# Autodesk Inventor assembly: Box
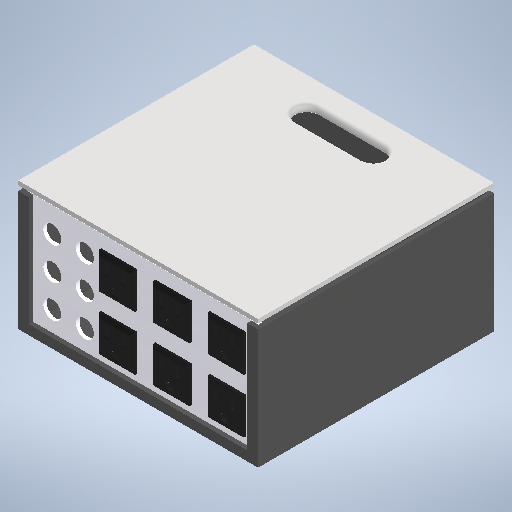
[picture p0: Inventor's stored thumbnail of the model, 512x512]
Saved by Autodesk Inventor 2025 (Build 290162000, 162)
## iProperties
Created: 2024-08-10
Part Number: Box
Document SubType Name: Assembly
Designer: ethan
Author: ethan
## Documents named in this file (5)
- C:\Users\ethan\Documents\GitHub\3D-Pants\AutoFrog\Box.iam
- C:\Users\ethan\Documents\GitHub\3D-Pants\AutoFrog\Box.ipt
- C:\Users\ethan\Documents\GitHub\3D-Pants\AutoFrog\faceplate.ipt
- C:\Users\ethan\Documents\GitHub\3D-Pants\AutoFrog\Plug.ipt
- C:\Users\ethan\Documents\GitHub\3D-Pants\AutoFrog\Lid.ipt
## Components (9 placed, 4 different names)
1. Box:1 — Mate:1, Mate:2, Flush:1, Flush:2
2. faceplate:1 — Mate:1, Mate:2, Mate:3, Mate:5, Mate:6, Mate:7, Mate:8, Mate:9, Mate:10, Mate:11, Mate:12, Mate:13, Mate:14, Mate:15, Mate:16, Mate:17, Mate:18, Mate:19, Mate:20, Mate:21, Mate:22
3. Plug:1 — Mate:8, Mate:9, Mate:10
4. Plug:2 — Mate:5, Mate:11, Mate:19
5. Plug:3 — Mate:7, Mate:13, Mate:18
6. Plug:4 — Mate:14, Mate:17, Mate:21
7. Plug:5 — Mate:6, Mate:15, Mate:16, Mate:22
8. Plug:6 — Mate:3, Mate:12, Mate:20
9. Lid:1 — Flush:1, Flush:2
## Relationships (23: Mate 21, Flush 2)
- Mate:1: Box:1 ↔ faceplate:1
- Mate:2: Box:1 ↔ faceplate:1
- Mate:3: faceplate:1 ↔ Plug:6
- Mate:5: faceplate:1 ↔ Plug:2
- Mate:6: faceplate:1 ↔ Plug:5
- Mate:7: faceplate:1 ↔ Plug:3
- Mate:8: faceplate:1 ↔ Plug:1
- Mate:9: faceplate:1 ↔ Plug:1
- Mate:10: faceplate:1 ↔ Plug:1
- Mate:11: faceplate:1 ↔ Plug:2
- Mate:12: faceplate:1 ↔ Plug:6
- Mate:13: faceplate:1 ↔ Plug:3
- Mate:14: faceplate:1 ↔ Plug:4
- Mate:15: faceplate:1 ↔ Plug:5
- Mate:16: faceplate:1 ↔ Plug:5
- Mate:17: faceplate:1 ↔ Plug:4
- Mate:18: faceplate:1 ↔ Plug:3
- Mate:19: faceplate:1 ↔ Plug:2
- Mate:20: faceplate:1 ↔ Plug:6
- Mate:21: faceplate:1 ↔ Plug:4
- Mate:22: faceplate:1 ↔ Plug:5
- Flush:1: Box:1 ↔ Lid:1
- Flush:2: Box:1 ↔ Lid:1
